# Autodesk Inventor assembly: Robot
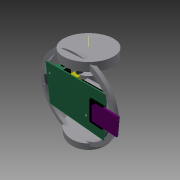
[picture p0: Inventor's stored thumbnail of the model, 180x180]
Saved by Autodesk Inventor 2014 (Build 180170000, 170)
## iProperties
Created: 2013-05-24
Part Number: Robot
Document SubType Name: Assembly
Designer: hartmann
Author: hartmann
## Documents named in this file (5)
- C:\Dokumente und Einstellungen\hartmann\Desktop\Robot\Robot.iam
- C:\Dokumente und Einstellungen\hartmann\Desktop\RaspberryPi\RaspberryPi.iam
- C:\Dokumente und Einstellungen\hartmann\Desktop\Robot\frame.ipt
- C:\Dokumente und Einstellungen\hartmann\Desktop\Robot\BaneBots2375.ipt
- C:\Dokumente und Einstellungen\hartmann\Desktop\Beep\Hardware\Model1\motor.ipt
## Components (6 placed, 4 different names)
1. RaspberryPi:1 [sub-assembly] — Fluchtend:1
2. frame:1 — Fluchtend:1
3. BaneBots2375:1 — Passend:1, Passend:2
4. BaneBots2375:2 — Passend:1, Passend:3
5. motor:1 — Passend:2, Passend:4
6. motor:2 — Passend:3, Passend:4
## Relationships (5: Mate 4, Flush 1)
- Fluchtend:1 [Flush]: RaspberryPi:1 ↔ frame:1
- Passend:1 [Mate]: BaneBots2375:1 ↔ BaneBots2375:2
- Passend:2 [Mate]: BaneBots2375:1 ↔ motor:1
- Passend:3 [Mate]: BaneBots2375:2 ↔ motor:2
- Passend:4 [Mate]: motor:1 ↔ motor:2
